# Autodesk Inventor assembly: multi-hotend-asm
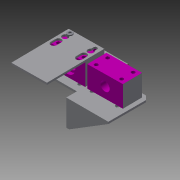
[picture p0: Inventor's stored thumbnail of the model, 180x180]
Saved by Autodesk Inventor 2014 (Build 180170000, 170)
## iProperties
Created: 2014-11-03
Part Number: multi-hotend-asm
Document SubType Name: Assembly
Designer: caleb
Author: caleb
## Documents named in this file (7)
- C:\cygwin\home\caleb\caleb-typea-settings\designs\bowden-extruder\multi-hotend-asm.iam
- C:\cygwin\home\caleb\caleb-typea-settings\designs\bowden-extruder\hotend_carrier.ipt
- C:\cygwin\home\caleb\caleb-typea-settings\designs\bowden-extruder\hotend holder rear.ipt
- C:\cygwin\home\caleb\caleb-typea-settings\designs\bowden-extruder\belt-grabber.ipt
- C:\cygwin\home\caleb\caleb-typea-settings\designs\bowden-extruder\Part2.ipt
- C:\Documents and Settings\caleb\My Documents\Inventor\Content Center Files\R2014\en-US\DIN 912\DIN 912 - M3 x 0.5 x 30 x 18.ipt
- C:\cygwin\home\caleb\caleb-typea-settings\designs\bowden-extruder\fan plenum.ipt
## Components (9 placed, 6 different names)
1. hotend_carrier:1 — Mate:1, Mate:2, Mate:3, Mate:10
2. hotend holder rear:1 — Flush:2, Mate:1, Mate:2, Mate:7, Mate:8, Mate:9, Mate:10, Flush:3
3. belt-grabber:1
4. Part2:1
5. hotend holder rear:2 — Flush:2, Mate:3, Mate:4, Mate:5, Mate:6, Flush:3
6. hotend holder rear:3 — Mate:7, Mate:8, Mate:9, Mate:11
7. hotend holder rear:4 — Mate:4, Mate:5, Mate:6, Mate:11, Mate:12, Mate:13
8. DIN 912 - replaced by DIN EN ISO 4762 M3 x 30:1 — Mate:12, Mate:13
9. fan plenum:1
## Relationships (15: Mate 13, Flush 2)
- Flush:2: hotend holder rear:1 ↔ hotend holder rear:2
- Mate:1: hotend_carrier:1 ↔ hotend holder rear:1
- Mate:2: hotend_carrier:1 ↔ hotend holder rear:1
- Mate:3: hotend_carrier:1 ↔ hotend holder rear:2
- Mate:4: hotend holder rear:2 ↔ hotend holder rear:4
- Mate:5: hotend holder rear:2 ↔ hotend holder rear:4
- Mate:6: hotend holder rear:2 ↔ hotend holder rear:4
- Mate:7 (31.302 mm): hotend holder rear:1 ↔ hotend holder rear:3
- Mate:8: hotend holder rear:1 ↔ hotend holder rear:3
- Mate:9: hotend holder rear:1 ↔ hotend holder rear:3
- Mate:10: hotend_carrier:1 ↔ hotend holder rear:1
- Mate:11: hotend holder rear:3 ↔ hotend holder rear:4
- Flush:3 (0.488 mm): hotend holder rear:1 ↔ hotend holder rear:2
- Mate:12: hotend holder rear:4 ↔ DIN 912 - replaced by DIN EN ISO 4762 M3 x 30:1
- Mate:13: hotend holder rear:4 ↔ DIN 912 - replaced by DIN EN ISO 4762 M3 x 30:1
